(part 1 of 2)
# Autodesk Inventor assembly: Display
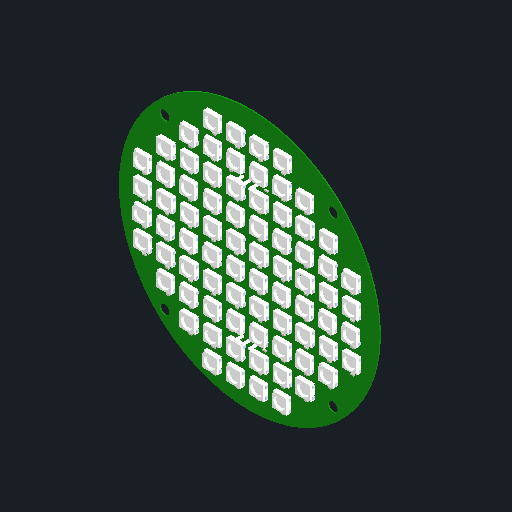
[picture p0: Inventor's stored thumbnail of the model, 512x512]
Saved by Autodesk Inventor 2026.2 (Build 302298000, 298)
## iProperties
Company: Open CASCADE
Created: 2026-06-05
Part Number: Display
Description: Open CASCADE Model
Document SubType Name: Assembly
Designer: User
Authority: Unknown
Title: Open CASCADE Shape Model
Author: Author
Sending System: Open CASCADE 7.5
Preprocessor: Open CASCADE STEP processor 7.5
## Documents named in this file (317)
- C:\Users\User\MyWorkspaces\DesktopBuddyRobot\BuddyRobot3DModel\Display\Display\Display.iam
- C:\Users\User\MyWorkspaces\DesktopBuddyRobot\BuddyRobot3DModel\Display\Display\Open CASCADE STEP translator 7.5 1.ipt
- C:\Users\User\MyWorkspaces\DesktopBuddyRobot\BuddyRobot3DModel\Display\Display\Open CASCADE STEP translator 7.5 2.ipt
- C:\Users\User\MyWorkspaces\DesktopBuddyRobot\BuddyRobot3DModel\Display\Display\Open CASCADE STEP translator 7.5 3.ipt
- C:\Users\User\MyWorkspaces\DesktopBuddyRobot\BuddyRobot3DModel\Display\Display\Open CASCADE STEP translator 7.5 4.ipt
- C:\Users\User\MyWorkspaces\DesktopBuddyRobot\BuddyRobot3DModel\Display\Display\Open CASCADE STEP translator 7.5 5.ipt
- C:\Users\User\MyWorkspaces\DesktopBuddyRobot\BuddyRobot3DModel\Display\Display\Open CASCADE STEP translator 7.5 6.ipt
- C:\Users\User\MyWorkspaces\DesktopBuddyRobot\BuddyRobot3DModel\Display\Display\Open CASCADE STEP translator 7.5 7.ipt
- C:\Users\User\MyWorkspaces\DesktopBuddyRobot\BuddyRobot3DModel\Display\Display\Open CASCADE STEP translator 7.5 8.ipt
- C:\Users\User\MyWorkspaces\DesktopBuddyRobot\BuddyRobot3DModel\Display\Display\Open CASCADE STEP translator 7.5 9.ipt
- C:\Users\User\MyWorkspaces\DesktopBuddyRobot\BuddyRobot3DModel\Display\Display\Open CASCADE STEP translator 7.5 10.ipt
- C:\Users\User\MyWorkspaces\DesktopBuddyRobot\BuddyRobot3DModel\Display\Display\Open CASCADE STEP translator 7.5 11.ipt
- C:\Users\User\MyWorkspaces\DesktopBuddyRobot\BuddyRobot3DModel\Display\Display\Open CASCADE STEP translator 7.5 12.ipt
- C:\Users\User\MyWorkspaces\DesktopBuddyRobot\BuddyRobot3DModel\Display\Display\Open CASCADE STEP translator 7.5 13.ipt
- C:\Users\User\MyWorkspaces\DesktopBuddyRobot\BuddyRobot3DModel\Display\Display\Open CASCADE STEP translator 7.5 14.ipt
- C:\Users\User\MyWorkspaces\DesktopBuddyRobot\BuddyRobot3DModel\Display\Display\Open CASCADE STEP translator 7.5 15.ipt
- C:\Users\User\MyWorkspaces\DesktopBuddyRobot\BuddyRobot3DModel\Display\Display\Open CASCADE STEP translator 7.5 16.ipt
- C:\Users\User\MyWorkspaces\DesktopBuddyRobot\BuddyRobot3DModel\Display\Display\Open CASCADE STEP translator 7.5 17.ipt
- C:\Users\User\MyWorkspaces\DesktopBuddyRobot\BuddyRobot3DModel\Display\Display\Open CASCADE STEP translator 7.5 18.ipt
- C:\Users\User\MyWorkspaces\DesktopBuddyRobot\BuddyRobot3DModel\Display\Display\Open CASCADE STEP translator 7.5 19.ipt
- C:\Users\User\MyWorkspaces\DesktopBuddyRobot\BuddyRobot3DModel\Display\Display\Open CASCADE STEP translator 7.5 20.ipt
- C:\Users\User\MyWorkspaces\DesktopBuddyRobot\BuddyRobot3DModel\Display\Display\Open CASCADE STEP translator 7.5 21.ipt
- C:\Users\User\MyWorkspaces\DesktopBuddyRobot\BuddyRobot3DModel\Display\Display\Open CASCADE STEP translator 7.5 22.ipt
- C:\Users\User\MyWorkspaces\DesktopBuddyRobot\BuddyRobot3DModel\Display\Display\Open CASCADE STEP translator 7.5 23.ipt
- C:\Users\User\MyWorkspaces\DesktopBuddyRobot\BuddyRobot3DModel\Display\Display\Open CASCADE STEP translator 7.5 24.ipt
- C:\Users\User\MyWorkspaces\DesktopBuddyRobot\BuddyRobot3DModel\Display\Display\Open CASCADE STEP translator 7.5 25.ipt
- C:\Users\User\MyWorkspaces\DesktopBuddyRobot\BuddyRobot3DModel\Display\Display\Open CASCADE STEP translator 7.5 26.ipt
- C:\Users\User\MyWorkspaces\DesktopBuddyRobot\BuddyRobot3DModel\Display\Display\Open CASCADE STEP translator 7.5 27.ipt
- C:\Users\User\MyWorkspaces\DesktopBuddyRobot\BuddyRobot3DModel\Display\Display\Open CASCADE STEP translator 7.5 28.ipt
- C:\Users\User\MyWorkspaces\DesktopBuddyRobot\BuddyRobot3DModel\Display\Display\Open CASCADE STEP translator 7.5 29.ipt
- C:\Users\User\MyWorkspaces\DesktopBuddyRobot\BuddyRobot3DModel\Display\Display\Open CASCADE STEP translator 7.5 30.ipt
- C:\Users\User\MyWorkspaces\DesktopBuddyRobot\BuddyRobot3DModel\Display\Display\Open CASCADE STEP translator 7.5 31.ipt
- C:\Users\User\MyWorkspaces\DesktopBuddyRobot\BuddyRobot3DModel\Display\Display\Open CASCADE STEP translator 7.5 32.ipt
- C:\Users\User\MyWorkspaces\DesktopBuddyRobot\BuddyRobot3DModel\Display\Display\Open CASCADE STEP translator 7.5 33.ipt
- C:\Users\User\MyWorkspaces\DesktopBuddyRobot\BuddyRobot3DModel\Display\Display\Open CASCADE STEP translator 7.5 34.ipt
- C:\Users\User\MyWorkspaces\DesktopBuddyRobot\BuddyRobot3DModel\Display\Display\Open CASCADE STEP translator 7.5 35.ipt
- C:\Users\User\MyWorkspaces\DesktopBuddyRobot\BuddyRobot3DModel\Display\Display\Open CASCADE STEP translator 7.5 36.ipt
- C:\Users\User\MyWorkspaces\DesktopBuddyRobot\BuddyRobot3DModel\Display\Display\Open CASCADE STEP translator 7.5 37.ipt
- C:\Users\User\MyWorkspaces\DesktopBuddyRobot\BuddyRobot3DModel\Display\Display\Open CASCADE STEP translator 7.5 38.ipt
- C:\Users\User\MyWorkspaces\DesktopBuddyRobot\BuddyRobot3DModel\Display\Display\Open CASCADE STEP translator 7.5 39.ipt
- C:\Users\User\MyWorkspaces\DesktopBuddyRobot\BuddyRobot3DModel\Display\Display\Open CASCADE STEP translator 7.5 40.ipt
- C:\Users\User\MyWorkspaces\DesktopBuddyRobot\BuddyRobot3DModel\Display\Display\Open CASCADE STEP translator 7.5 41.ipt
- C:\Users\User\MyWorkspaces\DesktopBuddyRobot\BuddyRobot3DModel\Display\Display\Open CASCADE STEP translator 7.5 42.ipt
- C:\Users\User\MyWorkspaces\DesktopBuddyRobot\BuddyRobot3DModel\Display\Display\Open CASCADE STEP translator 7.5 43.ipt
- C:\Users\User\MyWorkspaces\DesktopBuddyRobot\BuddyRobot3DModel\Display\Display\Open CASCADE STEP translator 7.5 44.ipt
- C:\Users\User\MyWorkspaces\DesktopBuddyRobot\BuddyRobot3DModel\Display\Display\Open CASCADE STEP translator 7.5 45.ipt
- C:\Users\User\MyWorkspaces\DesktopBuddyRobot\BuddyRobot3DModel\Display\Display\Open CASCADE STEP translator 7.5 46.ipt
- C:\Users\User\MyWorkspaces\DesktopBuddyRobot\BuddyRobot3DModel\Display\Display\Open CASCADE STEP translator 7.5 47.ipt
- C:\Users\User\MyWorkspaces\DesktopBuddyRobot\BuddyRobot3DModel\Display\Display\Open CASCADE STEP translator 7.5 48.ipt
- C:\Users\User\MyWorkspaces\DesktopBuddyRobot\BuddyRobot3DModel\Display\Display\Open CASCADE STEP translator 7.5 49.ipt
- C:\Users\User\MyWorkspaces\DesktopBuddyRobot\BuddyRobot3DModel\Display\Display\Open CASCADE STEP translator 7.5 50.ipt
- C:\Users\User\MyWorkspaces\DesktopBuddyRobot\BuddyRobot3DModel\Display\Display\Open CASCADE STEP translator 7.5 51.ipt
- C:\Users\User\MyWorkspaces\DesktopBuddyRobot\BuddyRobot3DModel\Display\Display\Open CASCADE STEP translator 7.5 52.ipt
- C:\Users\User\MyWorkspaces\DesktopBuddyRobot\BuddyRobot3DModel\Display\Display\Open CASCADE STEP translator 7.5 53.ipt
- C:\Users\User\MyWorkspaces\DesktopBuddyRobot\BuddyRobot3DModel\Display\Display\Open CASCADE STEP translator 7.5 54.ipt
- C:\Users\User\MyWorkspaces\DesktopBuddyRobot\BuddyRobot3DModel\Display\Display\Open CASCADE STEP translator 7.5 55.ipt
- C:\Users\User\MyWorkspaces\DesktopBuddyRobot\BuddyRobot3DModel\Display\Display\Open CASCADE STEP translator 7.5 56.ipt
- C:\Users\User\MyWorkspaces\DesktopBuddyRobot\BuddyRobot3DModel\Display\Display\Open CASCADE STEP translator 7.5 57.ipt
- C:\Users\User\MyWorkspaces\DesktopBuddyRobot\BuddyRobot3DModel\Display\Display\Open CASCADE STEP translator 7.5 58.ipt
- C:\Users\User\MyWorkspaces\DesktopBuddyRobot\BuddyRobot3DModel\Display\Display\Open CASCADE STEP translator 7.5 59.ipt
- C:\Users\User\MyWorkspaces\DesktopBuddyRobot\BuddyRobot3DModel\Display\Display\Open CASCADE STEP translator 7.5 60.ipt
- C:\Users\User\MyWorkspaces\DesktopBuddyRobot\BuddyRobot3DModel\Display\Display\Open CASCADE STEP translator 7.5 61.ipt
- C:\Users\User\MyWorkspaces\DesktopBuddyRobot\BuddyRobot3DModel\Display\Display\Open CASCADE STEP translator 7.5 62.ipt
- C:\Users\User\MyWorkspaces\DesktopBuddyRobot\BuddyRobot3DModel\Display\Display\Open CASCADE STEP translator 7.5 63.ipt
- C:\Users\User\MyWorkspaces\DesktopBuddyRobot\BuddyRobot3DModel\Display\Display\Open CASCADE STEP translator 7.5 64.ipt
- C:\Users\User\MyWorkspaces\DesktopBuddyRobot\BuddyRobot3DModel\Display\Display\Open CASCADE STEP translator 7.5 65.ipt
- C:\Users\User\MyWorkspaces\DesktopBuddyRobot\BuddyRobot3DModel\Display\Display\Open CASCADE STEP translator 7.5 66.ipt
- C:\Users\User\MyWorkspaces\DesktopBuddyRobot\BuddyRobot3DModel\Display\Display\Open CASCADE STEP translator 7.5 67.ipt
- C:\Users\User\MyWorkspaces\DesktopBuddyRobot\BuddyRobot3DModel\Display\Display\Open CASCADE STEP translator 7.5 68.ipt
- C:\Users\User\MyWorkspaces\DesktopBuddyRobot\BuddyRobot3DModel\Display\Display\Open CASCADE STEP translator 7.5 69.ipt
- C:\Users\User\MyWorkspaces\DesktopBuddyRobot\BuddyRobot3DModel\Display\Display\Open CASCADE STEP translator 7.5 70.ipt
- C:\Users\User\MyWorkspaces\DesktopBuddyRobot\BuddyRobot3DModel\Display\Display\Open CASCADE STEP translator 7.5 71.ipt
- C:\Users\User\MyWorkspaces\DesktopBuddyRobot\BuddyRobot3DModel\Display\Display\Open CASCADE STEP translator 7.5 72.ipt
- C:\Users\User\MyWorkspaces\DesktopBuddyRobot\BuddyRobot3DModel\Display\Display\Open CASCADE STEP translator 7.5 73.ipt
- C:\Users\User\MyWorkspaces\DesktopBuddyRobot\BuddyRobot3DModel\Display\Display\Open CASCADE STEP translator 7.5 74.ipt
- C:\Users\User\MyWorkspaces\DesktopBuddyRobot\BuddyRobot3DModel\Display\Display\Open CASCADE STEP translator 7.5 75.ipt
- C:\Users\User\MyWorkspaces\DesktopBuddyRobot\BuddyRobot3DModel\Display\Display\Open CASCADE STEP translator 7.5 76.ipt
- C:\Users\User\MyWorkspaces\DesktopBuddyRobot\BuddyRobot3DModel\Display\Display\Open CASCADE STEP translator 7.5 77.ipt
- C:\Users\User\MyWorkspaces\DesktopBuddyRobot\BuddyRobot3DModel\Display\Display\Open CASCADE STEP translator 7.5 78.ipt
- C:\Users\User\MyWorkspaces\DesktopBuddyRobot\BuddyRobot3DModel\Display\Display\Open CASCADE STEP translator 7.5 79.ipt
- C:\Users\User\MyWorkspaces\DesktopBuddyRobot\BuddyRobot3DModel\Display\Display\Open CASCADE STEP translator 7.5 80.ipt
- C:\Users\User\MyWorkspaces\DesktopBuddyRobot\BuddyRobot3DModel\Display\Display\Open CASCADE STEP translator 7.5 81.ipt
- C:\Users\User\MyWorkspaces\DesktopBuddyRobot\BuddyRobot3DModel\Display\Display\Open CASCADE STEP translator 7.5 82.ipt
- C:\Users\User\MyWorkspaces\DesktopBuddyRobot\BuddyRobot3DModel\Display\Display\Open CASCADE STEP translator 7.5 83.ipt
- C:\Users\User\MyWorkspaces\DesktopBuddyRobot\BuddyRobot3DModel\Display\Display\Open CASCADE STEP translator 7.5 84.ipt
- C:\Users\User\MyWorkspaces\DesktopBuddyRobot\BuddyRobot3DModel\Display\Display\Open CASCADE STEP translator 7.5 85.ipt
- C:\Users\User\MyWorkspaces\DesktopBuddyRobot\BuddyRobot3DModel\Display\Display\Open CASCADE STEP translator 7.5 86.ipt
- C:\Users\User\MyWorkspaces\DesktopBuddyRobot\BuddyRobot3DModel\Display\Display\Open CASCADE STEP translator 7.5 87.ipt
- C:\Users\User\MyWorkspaces\DesktopBuddyRobot\BuddyRobot3DModel\Display\Display\Open CASCADE STEP translator 7.5 88.ipt
- C:\Users\User\MyWorkspaces\DesktopBuddyRobot\BuddyRobot3DModel\Display\Display\Open CASCADE STEP translator 7.5 89.ipt
- C:\Users\User\MyWorkspaces\DesktopBuddyRobot\BuddyRobot3DModel\Display\Display\Open CASCADE STEP translator 7.5 90.ipt
- C:\Users\User\MyWorkspaces\DesktopBuddyRobot\BuddyRobot3DModel\Display\Display\Open CASCADE STEP translator 7.5 91.ipt
- C:\Users\User\MyWorkspaces\DesktopBuddyRobot\BuddyRobot3DModel\Display\Display\Open CASCADE STEP translator 7.5 92.ipt
- C:\Users\User\MyWorkspaces\DesktopBuddyRobot\BuddyRobot3DModel\Display\Display\Open CASCADE STEP translator 7.5 93.ipt
- C:\Users\User\MyWorkspaces\DesktopBuddyRobot\BuddyRobot3DModel\Display\Display\Open CASCADE STEP translator 7.5 94.ipt
- C:\Users\User\MyWorkspaces\DesktopBuddyRobot\BuddyRobot3DModel\Display\Display\Open CASCADE STEP translator 7.5 95.ipt
- C:\Users\User\MyWorkspaces\DesktopBuddyRobot\BuddyRobot3DModel\Display\Display\Open CASCADE STEP translator 7.5 96.ipt
- C:\Users\User\MyWorkspaces\DesktopBuddyRobot\BuddyRobot3DModel\Display\Display\Open CASCADE STEP translator 7.5 97.ipt
- C:\Users\User\MyWorkspaces\DesktopBuddyRobot\BuddyRobot3DModel\Display\Display\Open CASCADE STEP translator 7.5 98.ipt
- C:\Users\User\MyWorkspaces\DesktopBuddyRobot\BuddyRobot3DModel\Display\Display\Open CASCADE STEP translator 7.5 99.ipt
- C:\Users\User\MyWorkspaces\DesktopBuddyRobot\BuddyRobot3DModel\Display\Display\Open CASCADE STEP translator 7.5 100.ipt
- C:\Users\User\MyWorkspaces\DesktopBuddyRobot\BuddyRobot3DModel\Display\Display\Open CASCADE STEP translator 7.5 101.ipt
- C:\Users\User\MyWorkspaces\DesktopBuddyRobot\BuddyRobot3DModel\Display\Display\Open CASCADE STEP translator 7.5 102.ipt
- C:\Users\User\MyWorkspaces\DesktopBuddyRobot\BuddyRobot3DModel\Display\Display\Open CASCADE STEP translator 7.5 103.ipt
- C:\Users\User\MyWorkspaces\DesktopBuddyRobot\BuddyRobot3DModel\Display\Display\Open CASCADE STEP translator 7.5 104.ipt
- C:\Users\User\MyWorkspaces\DesktopBuddyRobot\BuddyRobot3DModel\Display\Display\Open CASCADE STEP translator 7.5 105.ipt
- C:\Users\User\MyWorkspaces\DesktopBuddyRobot\BuddyRobot3DModel\Display\Display\Open CASCADE STEP translator 7.5 106.ipt
- C:\Users\User\MyWorkspaces\DesktopBuddyRobot\BuddyRobot3DModel\Display\Display\Open CASCADE STEP translator 7.5 107.ipt
- C:\Users\User\MyWorkspaces\DesktopBuddyRobot\BuddyRobot3DModel\Display\Display\Open CASCADE STEP translator 7.5 108.ipt
- C:\Users\User\MyWorkspaces\DesktopBuddyRobot\BuddyRobot3DModel\Display\Display\Open CASCADE STEP translator 7.5 109.ipt
- C:\Users\User\MyWorkspaces\DesktopBuddyRobot\BuddyRobot3DModel\Display\Display\Open CASCADE STEP translator 7.5 110.ipt
- C:\Users\User\MyWorkspaces\DesktopBuddyRobot\BuddyRobot3DModel\Display\Display\Open CASCADE STEP translator 7.5 111.ipt
- C:\Users\User\MyWorkspaces\DesktopBuddyRobot\BuddyRobot3DModel\Display\Display\Open CASCADE STEP translator 7.5 112.ipt
- C:\Users\User\MyWorkspaces\DesktopBuddyRobot\BuddyRobot3DModel\Display\Display\Open CASCADE STEP translator 7.5 113.ipt
- C:\Users\User\MyWorkspaces\DesktopBuddyRobot\BuddyRobot3DModel\Display\Display\Open CASCADE STEP translator 7.5 114.ipt
- C:\Users\User\MyWorkspaces\DesktopBuddyRobot\BuddyRobot3DModel\Display\Display\Open CASCADE STEP translator 7.5 115.ipt
- C:\Users\User\MyWorkspaces\DesktopBuddyRobot\BuddyRobot3DModel\Display\Display\Open CASCADE STEP translator 7.5 116.ipt
- C:\Users\User\MyWorkspaces\DesktopBuddyRobot\BuddyRobot3DModel\Display\Display\Open CASCADE STEP translator 7.5 117.ipt
- C:\Users\User\MyWorkspaces\DesktopBuddyRobot\BuddyRobot3DModel\Display\Display\Open CASCADE STEP translator 7.5 118.ipt
- C:\Users\User\MyWorkspaces\DesktopBuddyRobot\BuddyRobot3DModel\Display\Display\Open CASCADE STEP translator 7.5 119.ipt
- C:\Users\User\MyWorkspaces\DesktopBuddyRobot\BuddyRobot3DModel\Display\Display\Open CASCADE STEP translator 7.5 120.ipt
- C:\Users\User\MyWorkspaces\DesktopBuddyRobot\BuddyRobot3DModel\Display\Display\Open CASCADE STEP translator 7.5 121.ipt
- C:\Users\User\MyWorkspaces\DesktopBuddyRobot\BuddyRobot3DModel\Display\Display\Open CASCADE STEP translator 7.5 122.ipt
- C:\Users\User\MyWorkspaces\DesktopBuddyRobot\BuddyRobot3DModel\Display\Display\Open CASCADE STEP translator 7.5 123.ipt
- C:\Users\User\MyWorkspaces\DesktopBuddyRobot\BuddyRobot3DModel\Display\Display\Open CASCADE STEP translator 7.5 124.ipt
- C:\Users\User\MyWorkspaces\DesktopBuddyRobot\BuddyRobot3DModel\Display\Display\Open CASCADE STEP translator 7.5 125.ipt
- C:\Users\User\MyWorkspaces\DesktopBuddyRobot\BuddyRobot3DModel\Display\Display\Open CASCADE STEP translator 7.5 126.ipt
- C:\Users\User\MyWorkspaces\DesktopBuddyRobot\BuddyRobot3DModel\Display\Display\Open CASCADE STEP translator 7.5 127.ipt
- C:\Users\User\MyWorkspaces\DesktopBuddyRobot\BuddyRobot3DModel\Display\Display\Open CASCADE STEP translator 7.5 128.ipt
- C:\Users\User\MyWorkspaces\DesktopBuddyRobot\BuddyRobot3DModel\Display\Display\Open CASCADE STEP translator 7.5 129.ipt
- C:\Users\User\MyWorkspaces\DesktopBuddyRobot\BuddyRobot3DModel\Display\Display\Open CASCADE STEP translator 7.5 130.ipt
- C:\Users\User\MyWorkspaces\DesktopBuddyRobot\BuddyRobot3DModel\Display\Display\Open CASCADE STEP translator 7.5 131.ipt
- C:\Users\User\MyWorkspaces\DesktopBuddyRobot\BuddyRobot3DModel\Display\Display\Open CASCADE STEP translator 7.5 132.ipt
- C:\Users\User\MyWorkspaces\DesktopBuddyRobot\BuddyRobot3DModel\Display\Display\Open CASCADE STEP translator 7.5 133.ipt
- C:\Users\User\MyWorkspaces\DesktopBuddyRobot\BuddyRobot3DModel\Display\Display\Open CASCADE STEP translator 7.5 134.ipt
- C:\Users\User\MyWorkspaces\DesktopBuddyRobot\BuddyRobot3DModel\Display\Display\Open CASCADE STEP translator 7.5 135.ipt
- C:\Users\User\MyWorkspaces\DesktopBuddyRobot\BuddyRobot3DModel\Display\Display\Open CASCADE STEP translator 7.5 136.ipt
- C:\Users\User\MyWorkspaces\DesktopBuddyRobot\BuddyRobot3DModel\Display\Display\Open CASCADE STEP translator 7.5 137.ipt
- C:\Users\User\MyWorkspaces\DesktopBuddyRobot\BuddyRobot3DModel\Display\Display\Open CASCADE STEP translator 7.5 138.ipt
- C:\Users\User\MyWorkspaces\DesktopBuddyRobot\BuddyRobot3DModel\Display\Display\Open CASCADE STEP translator 7.5 139.ipt
- C:\Users\User\MyWorkspaces\DesktopBuddyRobot\BuddyRobot3DModel\Display\Display\Open CASCADE STEP translator 7.5 140.ipt
- C:\Users\User\MyWorkspaces\DesktopBuddyRobot\BuddyRobot3DModel\Display\Display\Open CASCADE STEP translator 7.5 141.ipt
- C:\Users\User\MyWorkspaces\DesktopBuddyRobot\BuddyRobot3DModel\Display\Display\Open CASCADE STEP translator 7.5 142.ipt
- C:\Users\User\MyWorkspaces\DesktopBuddyRobot\BuddyRobot3DModel\Display\Display\Open CASCADE STEP translator 7.5 143.ipt
- C:\Users\User\MyWorkspaces\DesktopBuddyRobot\BuddyRobot3DModel\Display\Display\Open CASCADE STEP translator 7.5 144.ipt
- C:\Users\User\MyWorkspaces\DesktopBuddyRobot\BuddyRobot3DModel\Display\Display\Open CASCADE STEP translator 7.5 145.ipt
- C:\Users\User\MyWorkspaces\DesktopBuddyRobot\BuddyRobot3DModel\Display\Display\Open CASCADE STEP translator 7.5 146.ipt
- C:\Users\User\MyWorkspaces\DesktopBuddyRobot\BuddyRobot3DModel\Display\Display\Open CASCADE STEP translator 7.5 147.ipt
- C:\Users\User\MyWorkspaces\DesktopBuddyRobot\BuddyRobot3DModel\Display\Display\Open CASCADE STEP translator 7.5 148.ipt
- C:\Users\User\MyWorkspaces\DesktopBuddyRobot\BuddyRobot3DModel\Display\Display\Open CASCADE STEP translator 7.5 149.ipt
- C:\Users\User\MyWorkspaces\DesktopBuddyRobot\BuddyRobot3DModel\Display\Display\Open CASCADE STEP translator 7.5 150.ipt
- C:\Users\User\MyWorkspaces\DesktopBuddyRobot\BuddyRobot3DModel\Display\Display\Open CASCADE STEP translator 7.5 151.ipt
- C:\Users\User\MyWorkspaces\DesktopBuddyRobot\BuddyRobot3DModel\Display\Display\Open CASCADE STEP translator 7.5 152.ipt
- C:\Users\User\MyWorkspaces\DesktopBuddyRobot\BuddyRobot3DModel\Display\Display\Open CASCADE STEP translator 7.5 153.ipt
- C:\Users\User\MyWorkspaces\DesktopBuddyRobot\BuddyRobot3DModel\Display\Display\Open CASCADE STEP translator 7.5 154.ipt
- C:\Users\User\MyWorkspaces\DesktopBuddyRobot\BuddyRobot3DModel\Display\Display\Open CASCADE STEP translator 7.5 155.ipt
- C:\Users\User\MyWorkspaces\DesktopBuddyRobot\BuddyRobot3DModel\Display\Display\Open CASCADE STEP translator 7.5 156.ipt
- C:\Users\User\MyWorkspaces\DesktopBuddyRobot\BuddyRobot3DModel\Display\Display\Open CASCADE STEP translator 7.5 157.ipt
- C:\Users\User\MyWorkspaces\DesktopBuddyRobot\BuddyRobot3DModel\Display\Display\Open CASCADE STEP translator 7.5 158.ipt
- C:\Users\User\MyWorkspaces\DesktopBuddyRobot\BuddyRobot3DModel\Display\Display\Open CASCADE STEP translator 7.5 159.ipt
- C:\Users\User\MyWorkspaces\DesktopBuddyRobot\BuddyRobot3DModel\Display\Display\Open CASCADE STEP translator 7.5 160.ipt
- C:\Users\User\MyWorkspaces\DesktopBuddyRobot\BuddyRobot3DModel\Display\Display\Open CASCADE STEP translator 7.5 161.ipt
- C:\Users\User\MyWorkspaces\DesktopBuddyRobot\BuddyRobot3DModel\Display\Display\Open CASCADE STEP translator 7.5 162.ipt
- C:\Users\User\MyWorkspaces\DesktopBuddyRobot\BuddyRobot3DModel\Display\Display\Open CASCADE STEP translator 7.5 163.ipt
- C:\Users\User\MyWorkspaces\DesktopBuddyRobot\BuddyRobot3DModel\Display\Display\Open CASCADE STEP translator 7.5 164.ipt
- C:\Users\User\MyWorkspaces\DesktopBuddyRobot\BuddyRobot3DModel\Display\Display\Open CASCADE STEP translator 7.5 165.ipt
- C:\Users\User\MyWorkspaces\DesktopBuddyRobot\BuddyRobot3DModel\Display\Display\Open CASCADE STEP translator 7.5 166.ipt
- C:\Users\User\MyWorkspaces\DesktopBuddyRobot\BuddyRobot3DModel\Display\Display\Open CASCADE STEP translator 7.5 167.ipt
- C:\Users\User\MyWorkspaces\DesktopBuddyRobot\BuddyRobot3DModel\Display\Display\Open CASCADE STEP translator 7.5 168.ipt
- C:\Users\User\MyWorkspaces\DesktopBuddyRobot\BuddyRobot3DModel\Display\Display\Open CASCADE STEP translator 7.5 169.ipt
- C:\Users\User\MyWorkspaces\DesktopBuddyRobot\BuddyRobot3DModel\Display\Display\Open CASCADE STEP translator 7.5 170.ipt
- C:\Users\User\MyWorkspaces\DesktopBuddyRobot\BuddyRobot3DModel\Display\Display\Open CASCADE STEP translator 7.5 171.ipt
- C:\Users\User\MyWorkspaces\DesktopBuddyRobot\BuddyRobot3DModel\Display\Display\Open CASCADE STEP translator 7.5 172.ipt
- C:\Users\User\MyWorkspaces\DesktopBuddyRobot\BuddyRobot3DModel\Display\Display\Open CASCADE STEP translator 7.5 173.ipt
- C:\Users\User\MyWorkspaces\DesktopBuddyRobot\BuddyRobot3DModel\Display\Display\Open CASCADE STEP translator 7.5 174.ipt
- C:\Users\User\MyWorkspaces\DesktopBuddyRobot\BuddyRobot3DModel\Display\Display\Open CASCADE STEP translator 7.5 175.ipt
- C:\Users\User\MyWorkspaces\DesktopBuddyRobot\BuddyRobot3DModel\Display\Display\Open CASCADE STEP translator 7.5 176.ipt
- C:\Users\User\MyWorkspaces\DesktopBuddyRobot\BuddyRobot3DModel\Display\Display\Open CASCADE STEP translator 7.5 177.ipt
- C:\Users\User\MyWorkspaces\DesktopBuddyRobot\BuddyRobot3DModel\Display\Display\Open CASCADE STEP translator 7.5 178.ipt
- C:\Users\User\MyWorkspaces\DesktopBuddyRobot\BuddyRobot3DModel\Display\Display\Open CASCADE STEP translator 7.5 179.ipt
- C:\Users\User\MyWorkspaces\DesktopBuddyRobot\BuddyRobot3DModel\Display\Display\Open CASCADE STEP translator 7.5 180.ipt
- C:\Users\User\MyWorkspaces\DesktopBuddyRobot\BuddyRobot3DModel\Display\Display\Open CASCADE STEP translator 7.5 181.ipt
- C:\Users\User\MyWorkspaces\DesktopBuddyRobot\BuddyRobot3DModel\Display\Display\Open CASCADE STEP translator 7.5 182.ipt
- C:\Users\User\MyWorkspaces\DesktopBuddyRobot\BuddyRobot3DModel\Display\Display\Open CASCADE STEP translator 7.5 183.ipt
- C:\Users\User\MyWorkspaces\DesktopBuddyRobot\BuddyRobot3DModel\Display\Display\Open CASCADE STEP translator 7.5 184.ipt
- C:\Users\User\MyWorkspaces\DesktopBuddyRobot\BuddyRobot3DModel\Display\Display\Open CASCADE STEP translator 7.5 185.ipt
- C:\Users\User\MyWorkspaces\DesktopBuddyRobot\BuddyRobot3DModel\Display\Display\Open CASCADE STEP translator 7.5 186.ipt
- C:\Users\User\MyWorkspaces\DesktopBuddyRobot\BuddyRobot3DModel\Display\Display\Open CASCADE STEP translator 7.5 187.ipt
- C:\Users\User\MyWorkspaces\DesktopBuddyRobot\BuddyRobot3DModel\Display\Display\Open CASCADE STEP translator 7.5 188.ipt
- C:\Users\User\MyWorkspaces\DesktopBuddyRobot\BuddyRobot3DModel\Display\Display\Open CASCADE STEP translator 7.5 189.ipt
- C:\Users\User\MyWorkspaces\DesktopBuddyRobot\BuddyRobot3DModel\Display\Display\Open CASCADE STEP translator 7.5 190.ipt
- C:\Users\User\MyWorkspaces\DesktopBuddyRobot\BuddyRobot3DModel\Display\Display\Open CASCADE STEP translator 7.5 191.ipt
- C:\Users\User\MyWorkspaces\DesktopBuddyRobot\BuddyRobot3DModel\Display\Display\Open CASCADE STEP translator 7.5 192.ipt
- C:\Users\User\MyWorkspaces\DesktopBuddyRobot\BuddyRobot3DModel\Display\Display\Open CASCADE STEP translator 7.5 193.ipt
- C:\Users\User\MyWorkspaces\DesktopBuddyRobot\BuddyRobot3DModel\Display\Display\Open CASCADE STEP translator 7.5 194.ipt
- C:\Users\User\MyWorkspaces\DesktopBuddyRobot\BuddyRobot3DModel\Display\Display\Open CASCADE STEP translator 7.5 195.ipt
- C:\Users\User\MyWorkspaces\DesktopBuddyRobot\BuddyRobot3DModel\Display\Display\Open CASCADE STEP translator 7.5 196.ipt
- C:\Users\User\MyWorkspaces\DesktopBuddyRobot\BuddyRobot3DModel\Display\Display\Open CASCADE STEP translator 7.5 197.ipt
- C:\Users\User\MyWorkspaces\DesktopBuddyRobot\BuddyRobot3DModel\Display\Display\Open CASCADE STEP translator 7.5 198.ipt
- C:\Users\User\MyWorkspaces\DesktopBuddyRobot\BuddyRobot3DModel\Display\Display\Open CASCADE STEP translator 7.5 199.ipt
- C:\Users\User\MyWorkspaces\DesktopBuddyRobot\BuddyRobot3DModel\Display\Display\Open CASCADE STEP translator 7.5 200.ipt
- C:\Users\User\MyWorkspaces\DesktopBuddyRobot\BuddyRobot3DModel\Display\Display\Open CASCADE STEP translator 7.5 201.ipt
- C:\Users\User\MyWorkspaces\DesktopBuddyRobot\BuddyRobot3DModel\Display\Display\Open CASCADE STEP translator 7.5 202.ipt
- C:\Users\User\MyWorkspaces\DesktopBuddyRobot\BuddyRobot3DModel\Display\Display\Open CASCADE STEP translator 7.5 203.ipt
- C:\Users\User\MyWorkspaces\DesktopBuddyRobot\BuddyRobot3DModel\Display\Display\Open CASCADE STEP translator 7.5 204.ipt
- C:\Users\User\MyWorkspaces\DesktopBuddyRobot\BuddyRobot3DModel\Display\Display\Open CASCADE STEP translator 7.5 205.ipt
- C:\Users\User\MyWorkspaces\DesktopBuddyRobot\BuddyRobot3DModel\Display\Display\Open CASCADE STEP translator 7.5 206.ipt
- C:\Users\User\MyWorkspaces\DesktopBuddyRobot\BuddyRobot3DModel\Display\Display\Open CASCADE STEP translator 7.5 207.ipt
- C:\Users\User\MyWorkspaces\DesktopBuddyRobot\BuddyRobot3DModel\Display\Display\Open CASCADE STEP translator 7.5 208.ipt
- C:\Users\User\MyWorkspaces\DesktopBuddyRobot\BuddyRobot3DModel\Display\Display\Open CASCADE STEP translator 7.5 209.ipt
- C:\Users\User\MyWorkspaces\DesktopBuddyRobot\BuddyRobot3DModel\Display\Display\Open CASCADE STEP translator 7.5 210.ipt
- C:\Users\User\MyWorkspaces\DesktopBuddyRobot\BuddyRobot3DModel\Display\Display\Open CASCADE STEP translator 7.5 211.ipt
- C:\Users\User\MyWorkspaces\DesktopBuddyRobot\BuddyRobot3DModel\Display\Display\Open CASCADE STEP translator 7.5 212.ipt
- C:\Users\User\MyWorkspaces\DesktopBuddyRobot\BuddyRobot3DModel\Display\Display\Open CASCADE STEP translator 7.5 213.ipt
- C:\Users\User\MyWorkspaces\DesktopBuddyRobot\BuddyRobot3DModel\Display\Display\Open CASCADE STEP translator 7.5 214.ipt
- C:\Users\User\MyWorkspaces\DesktopBuddyRobot\BuddyRobot3DModel\Display\Display\Open CASCADE STEP translator 7.5 215.ipt
- C:\Users\User\MyWorkspaces\DesktopBuddyRobot\BuddyRobot3DModel\Display\Display\Open CASCADE STEP translator 7.5 216.ipt
- C:\Users\User\MyWorkspaces\DesktopBuddyRobot\BuddyRobot3DModel\Display\Display\Open CASCADE STEP translator 7.5 217.ipt
- C:\Users\User\MyWorkspaces\DesktopBuddyRobot\BuddyRobot3DModel\Display\Display\Open CASCADE STEP translator 7.5 218.ipt
- C:\Users\User\MyWorkspaces\DesktopBuddyRobot\BuddyRobot3DModel\Display\Display\Open CASCADE STEP translator 7.5 219.ipt
- C:\Users\User\MyWorkspaces\DesktopBuddyRobot\BuddyRobot3DModel\Display\Display\Open CASCADE STEP translator 7.5 220.ipt
- C:\Users\User\MyWorkspaces\DesktopBuddyRobot\BuddyRobot3DModel\Display\Display\Open CASCADE STEP translator 7.5 221.ipt
- C:\Users\User\MyWorkspaces\DesktopBuddyRobot\BuddyRobot3DModel\Display\Display\Open CASCADE STEP translator 7.5 222.ipt
- C:\Users\User\MyWorkspaces\DesktopBuddyRobot\BuddyRobot3DModel\Display\Display\Open CASCADE STEP translator 7.5 223.ipt
- C:\Users\User\MyWorkspaces\DesktopBuddyRobot\BuddyRobot3DModel\Display\Display\Open CASCADE STEP translator 7.5 224.ipt
- C:\Users\User\MyWorkspaces\DesktopBuddyRobot\BuddyRobot3DModel\Display\Display\Open CASCADE STEP translator 7.5 225.ipt
- C:\Users\User\MyWorkspaces\DesktopBuddyRobot\BuddyRobot3DModel\Display\Display\Open CASCADE STEP translator 7.5 226.ipt
- C:\Users\User\MyWorkspaces\DesktopBuddyRobot\BuddyRobot3DModel\Display\Display\Open CASCADE STEP translator 7.5 227.ipt
- C:\Users\User\MyWorkspaces\DesktopBuddyRobot\BuddyRobot3DModel\Display\Display\Open CASCADE STEP translator 7.5 228.ipt
- C:\Users\User\MyWorkspaces\DesktopBuddyRobot\BuddyRobot3DModel\Display\Display\Open CASCADE STEP translator 7.5 229.ipt
- C:\Users\User\MyWorkspaces\DesktopBuddyRobot\BuddyRobot3DModel\Display\Display\Open CASCADE STEP translator 7.5 230.ipt
- C:\Users\User\MyWorkspaces\DesktopBuddyRobot\BuddyRobot3DModel\Display\Display\Open CASCADE STEP translator 7.5 231.ipt
- C:\Users\User\MyWorkspaces\DesktopBuddyRobot\BuddyRobot3DModel\Display\Display\Open CASCADE STEP translator 7.5 232.ipt
- C:\Users\User\MyWorkspaces\DesktopBuddyRobot\BuddyRobot3DModel\Display\Display\Open CASCADE STEP translator 7.5 233.ipt
- C:\Users\User\MyWorkspaces\DesktopBuddyRobot\BuddyRobot3DModel\Display\Display\Open CASCADE STEP translator 7.5 234.ipt
- C:\Users\User\MyWorkspaces\DesktopBuddyRobot\BuddyRobot3DModel\Display\Display\Open CASCADE STEP translator 7.5 235.ipt
- C:\Users\User\MyWorkspaces\DesktopBuddyRobot\BuddyRobot3DModel\Display\Display\Open CASCADE STEP translator 7.5 236.ipt
- C:\Users\User\MyWorkspaces\DesktopBuddyRobot\BuddyRobot3DModel\Display\Display\Open CASCADE STEP translator 7.5 237.ipt
- C:\Users\User\MyWorkspaces\DesktopBuddyRobot\BuddyRobot3DModel\Display\Display\Open CASCADE STEP translator 7.5 238.ipt
- C:\Users\User\MyWorkspaces\DesktopBuddyRobot\BuddyRobot3DModel\Display\Display\Open CASCADE STEP translator 7.5 239.ipt
- C:\Users\User\MyWorkspaces\DesktopBuddyRobot\BuddyRobot3DModel\Display\Display\Open CASCADE STEP translator 7.5 240.ipt
- C:\Users\User\MyWorkspaces\DesktopBuddyRobot\BuddyRobot3DModel\Display\Display\Open CASCADE STEP translator 7.5 241.ipt
- C:\Users\User\MyWorkspaces\DesktopBuddyRobot\BuddyRobot3DModel\Display\Display\Open CASCADE STEP translator 7.5 242.ipt
- C:\Users\User\MyWorkspaces\DesktopBuddyRobot\BuddyRobot3DModel\Display\Display\Open CASCADE STEP translator 7.5 243.ipt
- C:\Users\User\MyWorkspaces\DesktopBuddyRobot\BuddyRobot3DModel\Display\Display\Open CASCADE STEP translator 7.5 244.ipt
- C:\Users\User\MyWorkspaces\DesktopBuddyRobot\BuddyRobot3DModel\Display\Display\Open CASCADE STEP translator 7.5 245.ipt
- C:\Users\User\MyWorkspaces\DesktopBuddyRobot\BuddyRobot3DModel\Display\Display\Open CASCADE STEP translator 7.5 246.ipt
- C:\Users\User\MyWorkspaces\DesktopBuddyRobot\BuddyRobot3DModel\Display\Display\Open CASCADE STEP translator 7.5 247.ipt
- C:\Users\User\MyWorkspaces\DesktopBuddyRobot\BuddyRobot3DModel\Display\Display\Open CASCADE STEP translator 7.5 248.ipt
- C:\Users\User\MyWorkspaces\DesktopBuddyRobot\BuddyRobot3DModel\Display\Display\Open CASCADE STEP translator 7.5 249.ipt
- C:\Users\User\MyWorkspaces\DesktopBuddyRobot\BuddyRobot3DModel\Display\Display\Open CASCADE STEP translator 7.5 250.ipt
- C:\Users\User\MyWorkspaces\DesktopBuddyRobot\BuddyRobot3DModel\Display\Display\Open CASCADE STEP translator 7.5 251.ipt
- C:\Users\User\MyWorkspaces\DesktopBuddyRobot\BuddyRobot3DModel\Display\Display\Open CASCADE STEP translator 7.5 252.ipt
- C:\Users\User\MyWorkspaces\DesktopBuddyRobot\BuddyRobot3DModel\Display\Display\Open CASCADE STEP translator 7.5 253.ipt
- C:\Users\User\MyWorkspaces\DesktopBuddyRobot\BuddyRobot3DModel\Display\Display\Open CASCADE STEP translator 7.5 254.ipt
- C:\Users\User\MyWorkspaces\DesktopBuddyRobot\BuddyRobot3DModel\Display\Display\Open CASCADE STEP translator 7.5 255.ipt
- C:\Users\User\MyWorkspaces\DesktopBuddyRobot\BuddyRobot3DModel\Display\Display\Open CASCADE STEP translator 7.5 256.ipt
- C:\Users\User\MyWorkspaces\DesktopBuddyRobot\BuddyRobot3DModel\Display\Display\Open CASCADE STEP translator 7.5 257.ipt
- C:\Users\User\MyWorkspaces\DesktopBuddyRobot\BuddyRobot3DModel\Display\Display\Open CASCADE STEP translator 7.5 258.ipt
- C:\Users\User\MyWorkspaces\DesktopBuddyRobot\BuddyRobot3DModel\Display\Display\Open CASCADE STEP translator 7.5 259.ipt
- C:\Users\User\MyWorkspaces\DesktopBuddyRobot\BuddyRobot3DModel\Display\Display\Open CASCADE STEP translator 7.5 260.ipt
- C:\Users\User\MyWorkspaces\DesktopBuddyRobot\BuddyRobot3DModel\Display\Display\Open CASCADE STEP translator 7.5 261.ipt
- C:\Users\User\MyWorkspaces\DesktopBuddyRobot\BuddyRobot3DModel\Display\Display\Open CASCADE STEP translator 7.5 262.ipt
- C:\Users\User\MyWorkspaces\DesktopBuddyRobot\BuddyRobot3DModel\Display\Display\Open CASCADE STEP translator 7.5 263.ipt
- C:\Users\User\MyWorkspaces\DesktopBuddyRobot\BuddyRobot3DModel\Display\Display\Open CASCADE STEP translator 7.5 264.ipt
- C:\Users\User\MyWorkspaces\DesktopBuddyRobot\BuddyRobot3DModel\Display\Display\Open CASCADE STEP translator 7.5 265.ipt
- C:\Users\User\MyWorkspaces\DesktopBuddyRobot\BuddyRobot3DModel\Display\Display\Open CASCADE STEP translator 7.5 266.ipt
- C:\Users\User\MyWorkspaces\DesktopBuddyRobot\BuddyRobot3DModel\Display\Display\Open CASCADE STEP translator 7.5 267.ipt
- C:\Users\User\MyWorkspaces\DesktopBuddyRobot\BuddyRobot3DModel\Display\Display\Open CASCADE STEP translator 7.5 268.ipt
- C:\Users\User\MyWorkspaces\DesktopBuddyRobot\BuddyRobot3DModel\Display\Display\Open CASCADE STEP translator 7.5 269.ipt
- C:\Users\User\MyWorkspaces\DesktopBuddyRobot\BuddyRobot3DModel\Display\Display\Open CASCADE STEP translator 7.5 270.ipt
- C:\Users\User\MyWorkspaces\DesktopBuddyRobot\BuddyRobot3DModel\Display\Display\Open CASCADE STEP translator 7.5 271.ipt
- C:\Users\User\MyWorkspaces\DesktopBuddyRobot\BuddyRobot3DModel\Display\Display\Open CASCADE STEP translator 7.5 272.ipt
- C:\Users\User\MyWorkspaces\DesktopBuddyRobot\BuddyRobot3DModel\Display\Display\Open CASCADE STEP translator 7.5 273.ipt
- C:\Users\User\MyWorkspaces\DesktopBuddyRobot\BuddyRobot3DModel\Display\Display\Open CASCADE STEP translator 7.5 274.ipt
- C:\Users\User\MyWorkspaces\DesktopBuddyRobot\BuddyRobot3DModel\Display\Display\Open CASCADE STEP translator 7.5 275.ipt
- C:\Users\User\MyWorkspaces\DesktopBuddyRobot\BuddyRobot3DModel\Display\Display\Open CASCADE STEP translator 7.5 276.ipt
- C:\Users\User\MyWorkspaces\DesktopBuddyRobot\BuddyRobot3DModel\Display\Display\Open CASCADE STEP translator 7.5 277.ipt
- C:\Users\User\MyWorkspaces\DesktopBuddyRobot\BuddyRobot3DModel\Display\Display\Open CASCADE STEP translator 7.5 278.ipt
- C:\Users\User\MyWorkspaces\DesktopBuddyRobot\BuddyRobot3DModel\Display\Display\Open CASCADE STEP translator 7.5 279.ipt
- C:\Users\User\MyWorkspaces\DesktopBuddyRobot\BuddyRobot3DModel\Display\Display\Open CASCADE STEP translator 7.5 280.ipt
- C:\Users\User\MyWorkspaces\DesktopBuddyRobot\BuddyRobot3DModel\Display\Display\Open CASCADE STEP translator 7.5 281.ipt
- C:\Users\User\MyWorkspaces\DesktopBuddyRobot\BuddyRobot3DModel\Display\Display\Open CASCADE STEP translator 7.5 282.ipt
- C:\Users\User\MyWorkspaces\DesktopBuddyRobot\BuddyRobot3DModel\Display\Display\Open CASCADE STEP translator 7.5 283.ipt
- C:\Users\User\MyWorkspaces\DesktopBuddyRobot\BuddyRobot3DModel\Display\Display\Open CASCADE STEP translator 7.5 284.ipt
- C:\Users\User\MyWorkspaces\DesktopBuddyRobot\BuddyRobot3DModel\Display\Display\Open CASCADE STEP translator 7.5 285.ipt
- C:\Users\User\MyWorkspaces\DesktopBuddyRobot\BuddyRobot3DModel\Display\Display\Open CASCADE STEP translator 7.5 286.ipt
- C:\Users\User\MyWorkspaces\DesktopBuddyRobot\BuddyRobot3DModel\Display\Display\Open CASCADE STEP translator 7.5 287.ipt
- C:\Users\User\MyWorkspaces\DesktopBuddyRobot\BuddyRobot3DModel\Display\Display\Open CASCADE STEP translator 7.5 288.ipt
- C:\Users\User\MyWorkspaces\DesktopBuddyRobot\BuddyRobot3DModel\Display\Display\Open CASCADE STEP translator 7.5 289.ipt
- C:\Users\User\MyWorkspaces\DesktopBuddyRobot\BuddyRobot3DModel\Display\Display\Open CASCADE STEP translator 7.5 290.ipt
- C:\Users\User\MyWorkspaces\DesktopBuddyRobot\BuddyRobot3DModel\Display\Display\Open CASCADE STEP translator 7.5 291.ipt
- C:\Users\User\MyWorkspaces\DesktopBuddyRobot\BuddyRobot3DModel\Display\Display\Open CASCADE STEP translator 7.5 292.ipt
- C:\Users\User\MyWorkspaces\DesktopBuddyRobot\BuddyRobot3DModel\Display\Display\Open CASCADE STEP translator 7.5 293.ipt
- C:\Users\User\MyWorkspaces\DesktopBuddyRobot\BuddyRobot3DModel\Display\Display\Open CASCADE STEP translator 7.5 294.ipt
- C:\Users\User\MyWorkspaces\DesktopBuddyRobot\BuddyRobot3DModel\Display\Display\Open CASCADE STEP translator 7.5 295.ipt
- C:\Users\User\MyWorkspaces\DesktopBuddyRobot\BuddyRobot3DModel\Display\Display\Open CASCADE STEP translator 7.5 296.ipt
- C:\Users\User\MyWorkspaces\DesktopBuddyRobot\BuddyRobot3DModel\Display\Display\Open CASCADE STEP translator 7.5 297.ipt
- C:\Users\User\MyWorkspaces\DesktopBuddyRobot\BuddyRobot3DModel\Display\Display\Open CASCADE STEP translator 7.5 298.ipt
- C:\Users\User\MyWorkspaces\DesktopBuddyRobot\BuddyRobot3DModel\Display\Display\Open CASCADE STEP translator 7.5 299.ipt
- C:\Users\User\MyWorkspaces\DesktopBuddyRobot\BuddyRobot3DModel\Display\Display\Open CASCADE STEP translator 7.5 300.ipt
- C:\Users\User\MyWorkspaces\DesktopBuddyRobot\BuddyRobot3DModel\Display\Display\Open CASCADE STEP translator 7.5 301.ipt
- C:\Users\User\MyWorkspaces\DesktopBuddyRobot\BuddyRobot3DModel\Display\Display\Open CASCADE STEP translator 7.5 302.ipt
- C:\Users\User\MyWorkspaces\DesktopBuddyRobot\BuddyRobot3DModel\Display\Display\Open CASCADE STEP translator 7.5 303.ipt
- C:\Users\User\MyWorkspaces\DesktopBuddyRobot\BuddyRobot3DModel\Display\Display\Open CASCADE STEP translator 7.5 304.ipt
- C:\Users\User\MyWorkspaces\DesktopBuddyRobot\BuddyRobot3DModel\Display\Display\Open CASCADE STEP translator 7.5 305.ipt
- C:\Users\User\MyWorkspaces\DesktopBuddyRobot\BuddyRobot3DModel\Display\Display\Open CASCADE STEP translator 7.5 306.ipt
- C:\Users\User\MyWorkspaces\DesktopBuddyRobot\BuddyRobot3DModel\Display\Display\Open CASCADE STEP translator 7.5 307.ipt
- C:\Users\User\MyWorkspaces\DesktopBuddyRobot\BuddyRobot3DModel\Display\Display\Open CASCADE STEP translator 7.5 308.ipt
- C:\Users\User\MyWorkspaces\DesktopBuddyRobot\BuddyRobot3DModel\Display\Display\Open CASCADE STEP translator 7.5 309.ipt
- C:\Users\User\MyWorkspaces\DesktopBuddyRobot\BuddyRobot3DModel\Display\Display\Open CASCADE STEP translator 7.5 310.ipt
- C:\Users\User\MyWorkspaces\DesktopBuddyRobot\BuddyRobot3DModel\Display\Display\Open CASCADE STEP translator 7.5 311.ipt
- C:\Users\User\MyWorkspaces\DesktopBuddyRobot\BuddyRobot3DModel\Display\Display\Open CASCADE STEP translator 7.5 312.ipt
- C:\Users\User\MyWorkspaces\DesktopBuddyRobot\BuddyRobot3DModel\Display\Display\Open CASCADE STEP translator 7.5 313.ipt
- C:\Users\User\MyWorkspaces\DesktopBuddyRobot\BuddyRobot3DModel\Display\Display\Open CASCADE STEP translator 7.5 314.ipt
- C:\Users\User\MyWorkspaces\DesktopBuddyRobot\BuddyRobot3DModel\Display\Display\Open CASCADE STEP translator 7.5 315.ipt
- C:\Users\User\MyWorkspaces\DesktopBuddyRobot\BuddyRobot3DModel\Display\Display\Open CASCADE STEP translator 7.5 316.ipt
## Components (316 placed, 316 different names)
1. Open CASCADE STEP translator 7.5 1
2. Open CASCADE STEP translator 7.5 2
3. Open CASCADE STEP translator 7.5 3
4. Open CASCADE STEP translator 7.5 4
5. Open CASCADE STEP translator 7.5 5
6. Open CASCADE STEP translator 7.5 6
7. Open CASCADE STEP translator 7.5 7
8. Open CASCADE STEP translator 7.5 8
9. Open CASCADE STEP translator 7.5 9
10. Open CASCADE STEP translator 7.5 10
11. Open CASCADE STEP translator 7.5 11
12. Open CASCADE STEP translator 7.5 12
13. Open CASCADE STEP translator 7.5 13
14. Open CASCADE STEP translator 7.5 14
15. Open CASCADE STEP translator 7.5 15
16. Open CASCADE STEP translator 7.5 16
17. Open CASCADE STEP translator 7.5 17
18. Open CASCADE STEP translator 7.5 18
19. Open CASCADE STEP translator 7.5 19
20. Open CASCADE STEP translator 7.5 20
21. Open CASCADE STEP translator 7.5 21
22. Open CASCADE STEP translator 7.5 22
23. Open CASCADE STEP translator 7.5 23
24. Open CASCADE STEP translator 7.5 24
25. Open CASCADE STEP translator 7.5 25
26. Open CASCADE STEP translator 7.5 26
27. Open CASCADE STEP translator 7.5 27
28. Open CASCADE STEP translator 7.5 28
29. Open CASCADE STEP translator 7.5 29
30. Open CASCADE STEP translator 7.5 30
31. Open CASCADE STEP translator 7.5 31
32. Open CASCADE STEP translator 7.5 32
33. Open CASCADE STEP translator 7.5 33
34. Open CASCADE STEP translator 7.5 34
35. Open CASCADE STEP translator 7.5 35
36. Open CASCADE STEP translator 7.5 36
37. Open CASCADE STEP translator 7.5 37
38. Open CASCADE STEP translator 7.5 38
39. Open CASCADE STEP translator 7.5 39
40. Open CASCADE STEP translator 7.5 40
41. Open CASCADE STEP translator 7.5 41
42. Open CASCADE STEP translator 7.5 42
43. Open CASCADE STEP translator 7.5 43
44. Open CASCADE STEP translator 7.5 44
45. Open CASCADE STEP translator 7.5 45
46. Open CASCADE STEP translator 7.5 46
47. Open CASCADE STEP translator 7.5 47
48. Open CASCADE STEP translator 7.5 48
49. Open CASCADE STEP translator 7.5 49
50. Open CASCADE STEP translator 7.5 50
51. Open CASCADE STEP translator 7.5 51
52. Open CASCADE STEP translator 7.5 52
53. Open CASCADE STEP translator 7.5 53
54. Open CASCADE STEP translator 7.5 54
55. Open CASCADE STEP translator 7.5 55
56. Open CASCADE STEP translator 7.5 56
57. Open CASCADE STEP translator 7.5 57
58. Open CASCADE STEP translator 7.5 58
59. Open CASCADE STEP translator 7.5 59
60. Open CASCADE STEP translator 7.5 60
61. Open CASCADE STEP translator 7.5 61
62. Open CASCADE STEP translator 7.5 62
63. Open CASCADE STEP translator 7.5 63
64. Open CASCADE STEP translator 7.5 64
65. Open CASCADE STEP translator 7.5 65
66. Open CASCADE STEP translator 7.5 66
67. Open CASCADE STEP translator 7.5 67
68. Open CASCADE STEP translator 7.5 68
69. Open CASCADE STEP translator 7.5 69
70. Open CASCADE STEP translator 7.5 70
71. Open CASCADE STEP translator 7.5 71
72. Open CASCADE STEP translator 7.5 72
73. Open CASCADE STEP translator 7.5 73
74. Open CASCADE STEP translator 7.5 74
75. Open CASCADE STEP translator 7.5 75
76. Open CASCADE STEP translator 7.5 76
77. Open CASCADE STEP translator 7.5 77
78. Open CASCADE STEP translator 7.5 78
79. Open CASCADE STEP translator 7.5 79
80. Open CASCADE STEP translator 7.5 80
81. Open CASCADE STEP translator 7.5 81
82. Open CASCADE STEP translator 7.5 82
83. Open CASCADE STEP translator 7.5 83
84. Open CASCADE STEP translator 7.5 84
85. Open CASCADE STEP translator 7.5 85
86. Open CASCADE STEP translator 7.5 86
87. Open CASCADE STEP translator 7.5 87
88. Open CASCADE STEP translator 7.5 88
89. Open CASCADE STEP translator 7.5 89
90. Open CASCADE STEP translator 7.5 90
91. Open CASCADE STEP translator 7.5 91
92. Open CASCADE STEP translator 7.5 92
93. Open CASCADE STEP translator 7.5 93
94. Open CASCADE STEP translator 7.5 94
95. Open CASCADE STEP translator 7.5 95
96. Open CASCADE STEP translator 7.5 96
97. Open CASCADE STEP translator 7.5 97
98. Open CASCADE STEP translator 7.5 98
99. Open CASCADE STEP translator 7.5 99
100. Open CASCADE STEP translator 7.5 100
101. Open CASCADE STEP translator 7.5 101
102. Open CASCADE STEP translator 7.5 102
103. Open CASCADE STEP translator 7.5 103
104. Open CASCADE STEP translator 7.5 104
105. Open CASCADE STEP translator 7.5 105
106. Open CASCADE STEP translator 7.5 106
107. Open CASCADE STEP translator 7.5 107
108. Open CASCADE STEP translator 7.5 108
109. Open CASCADE STEP translator 7.5 109
110. Open CASCADE STEP translator 7.5 110
111. Open CASCADE STEP translator 7.5 111
112. Open CASCADE STEP translator 7.5 112
113. Open CASCADE STEP translator 7.5 113
114. Open CASCADE STEP translator 7.5 114
115. Open CASCADE STEP translator 7.5 115
116. Open CASCADE STEP translator 7.5 116
117. Open CASCADE STEP translator 7.5 117
118. Open CASCADE STEP translator 7.5 118
119. Open CASCADE STEP translator 7.5 119
120. Open CASCADE STEP translator 7.5 120
121. Open CASCADE STEP translator 7.5 121
122. Open CASCADE STEP translator 7.5 122
123. Open CASCADE STEP translator 7.5 123
124. Open CASCADE STEP translator 7.5 124
125. Open CASCADE STEP translator 7.5 125
126. Open CASCADE STEP translator 7.5 126
127. Open CASCADE STEP translator 7.5 127
128. Open CASCADE STEP translator 7.5 128
129. Open CASCADE STEP translator 7.5 129
130. Open CASCADE STEP translator 7.5 130
131. Open CASCADE STEP translator 7.5 131
132. Open CASCADE STEP translator 7.5 132
133. Open CASCADE STEP translator 7.5 133
134. Open CASCADE STEP translator 7.5 134
135. Open CASCADE STEP translator 7.5 135
136. Open CASCADE STEP translator 7.5 136
137. Open CASCADE STEP translator 7.5 137
138. Open CASCADE STEP translator 7.5 138
139. Open CASCADE STEP translator 7.5 139
140. Open CASCADE STEP translator 7.5 140
141. Open CASCADE STEP translator 7.5 141
142. Open CASCADE STEP translator 7.5 142
143. Open CASCADE STEP translator 7.5 143
144. Open CASCADE STEP translator 7.5 144
145. Open CASCADE STEP translator 7.5 145
146. Open CASCADE STEP translator 7.5 146
147. Open CASCADE STEP translator 7.5 147
148. Open CASCADE STEP translator 7.5 148
149. Open CASCADE STEP translator 7.5 149
150. Open CASCADE STEP translator 7.5 150
151. Open CASCADE STEP translator 7.5 151
152. Open CASCADE STEP translator 7.5 152
153. Open CASCADE STEP translator 7.5 153
154. Open CASCADE STEP translator 7.5 154
155. Open CASCADE STEP translator 7.5 155
156. Open CASCADE STEP translator 7.5 156
157. Open CASCADE STEP translator 7.5 157
158. Open CASCADE STEP translator 7.5 158
159. Open CASCADE STEP translator 7.5 159
160. Open CASCADE STEP translator 7.5 160
161. Open CASCADE STEP translator 7.5 161
162. Open CASCADE STEP translator 7.5 162
163. Open CASCADE STEP translator 7.5 163
164. Open CASCADE STEP translator 7.5 164
165. Open CASCADE STEP translator 7.5 165
166. Open CASCADE STEP translator 7.5 166
167. Open CASCADE STEP translator 7.5 167
168. Open CASCADE STEP translator 7.5 168
169. Open CASCADE STEP translator 7.5 169
170. Open CASCADE STEP translator 7.5 170
171. Open CASCADE STEP translator 7.5 171
172. Open CASCADE STEP translator 7.5 172
173. Open CASCADE STEP translator 7.5 173
174. Open CASCADE STEP translator 7.5 174
175. Open CASCADE STEP translator 7.5 175
176. Open CASCADE STEP translator 7.5 176
177. Open CASCADE STEP translator 7.5 177
178. Open CASCADE STEP translator 7.5 178
179. Open CASCADE STEP translator 7.5 179
180. Open CASCADE STEP translator 7.5 180
181. Open CASCADE STEP translator 7.5 181
182. Open CASCADE STEP translator 7.5 182
183. Open CASCADE STEP translator 7.5 183
184. Open CASCADE STEP translator 7.5 184
185. Open CASCADE STEP translator 7.5 185
186. Open CASCADE STEP translator 7.5 186
187. Open CASCADE STEP translator 7.5 187
188. Open CASCADE STEP translator 7.5 188
189. Open CASCADE STEP translator 7.5 189
190. Open CASCADE STEP translator 7.5 190
191. Open CASCADE STEP translator 7.5 191
192. Open CASCADE STEP translator 7.5 192
193. Open CASCADE STEP translator 7.5 193
194. Open CASCADE STEP translator 7.5 194
195. Open CASCADE STEP translator 7.5 195
196. Open CASCADE STEP translator 7.5 196
197. Open CASCADE STEP translator 7.5 197
198. Open CASCADE STEP translator 7.5 198
199. Open CASCADE STEP translator 7.5 199
200. Open CASCADE STEP translator 7.5 200
201. Open CASCADE STEP translator 7.5 201
202. Open CASCADE STEP translator 7.5 202
203. Open CASCADE STEP translator 7.5 203
204. Open CASCADE STEP translator 7.5 204
205. Open CASCADE STEP translator 7.5 205
206. Open CASCADE STEP translator 7.5 206
207. Open CASCADE STEP translator 7.5 207
208. Open CASCADE STEP translator 7.5 208
209. Open CASCADE STEP translator 7.5 209
210. Open CASCADE STEP translator 7.5 210
211. Open CASCADE STEP translator 7.5 211
212. Open CASCADE STEP translator 7.5 212
213. Open CASCADE STEP translator 7.5 213
214. Open CASCADE STEP translator 7.5 214
215. Open CASCADE STEP translator 7.5 215
216. Open CASCADE STEP translator 7.5 216
217. Open CASCADE STEP translator 7.5 217
218. Open CASCADE STEP translator 7.5 218
219. Open CASCADE STEP translator 7.5 219
220. Open CASCADE STEP translator 7.5 220
221. Open CASCADE STEP translator 7.5 221
222. Open CASCADE STEP translator 7.5 222
223. Open CASCADE STEP translator 7.5 223
224. Open CASCADE STEP translator 7.5 224
225. Open CASCADE STEP translator 7.5 225
226. Open CASCADE STEP translator 7.5 226
227. Open CASCADE STEP translator 7.5 227
228. Open CASCADE STEP translator 7.5 228
229. Open CASCADE STEP translator 7.5 229
230. Open CASCADE STEP translator 7.5 230
231. Open CASCADE STEP translator 7.5 231
232. Open CASCADE STEP translator 7.5 232
233. Open CASCADE STEP translator 7.5 233
234. Open CASCADE STEP translator 7.5 234
235. Open CASCADE STEP translator 7.5 235
236. Open CASCADE STEP translator 7.5 236
237. Open CASCADE STEP translator 7.5 237
238. Open CASCADE STEP translator 7.5 238
239. Open CASCADE STEP translator 7.5 239
240. Open CASCADE STEP translator 7.5 240
241. Open CASCADE STEP translator 7.5 241
242. Open CASCADE STEP translator 7.5 242
243. Open CASCADE STEP translator 7.5 243
244. Open CASCADE STEP translator 7.5 244
245. Open CASCADE STEP translator 7.5 245
246. Open CASCADE STEP translator 7.5 246
247. Open CASCADE STEP translator 7.5 247
248. Open CASCADE STEP translator 7.5 248
249. Open CASCADE STEP translator 7.5 249
250. Open CASCADE STEP translator 7.5 250
251. Open CASCADE STEP translator 7.5 251
252. Open CASCADE STEP translator 7.5 252
253. Open CASCADE STEP translator 7.5 253
254. Open CASCADE STEP translator 7.5 254
255. Open CASCADE STEP translator 7.5 255
256. Open CASCADE STEP translator 7.5 256
257. Open CASCADE STEP translator 7.5 257
258. Open CASCADE STEP translator 7.5 258
259. Open CASCADE STEP translator 7.5 259
260. Open CASCADE STEP translator 7.5 260
261. Open CASCADE STEP translator 7.5 261
262. Open CASCADE STEP translator 7.5 262